# Autodesk Inventor assembly: GE-12022
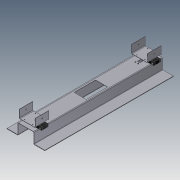
[picture p0: Inventor's stored thumbnail of the model, 180x180]
Saved by Autodesk Inventor 2012 (Build 160160000, 160)
## iProperties
Created: 2011-06-06
Part Number: GE-12022
Document SubType Name: Assembly
Designer: dfoster
Description: Base Assembly, Bridge
Title: Base Assembly, Bridge
Author: dfoster
## Documents named in this file (14)
- C:\Data Folder\FRC 2012 Field\Components\GE-12022.iam
- C:\Data Folder\FRC 2012 Field\Components\GE-12021.ipt
- C:\Data Folder\FRC 2012 Field\Components\PP-00065.ipt
- C:\Data Folder\FRC 2012 Field\Components\GE-12023.ipt
- C:\Data Folder\FRC 2012 Field\Components\GE-12024.ipt
- C:\Data Folder\FRC 2012 Field\Components\GE-12025.ipt
- C:\Data Folder\FRC 2012 Field\Components\HW-00043.0001.ipt
- C:\Data Folder\FRC 2012 Field\Components\HW-00064.ipt
- C:\Data Folder\FRC 2012 Field\Components\HW-00065.ipt
- C:\Data Folder\FRC 2012 Field\Components\HW-00033.ipt
- C:\Data Folder\FRC 2012 Field\Components\GE-12061.ipt
- C:\Data Folder\FRC 2012 Field\Components\HW-00070.ipt
- C:\Data Folder\FRC 2012 Field\Components\HW-00071.ipt
- C:\Data Folder\FRC 2012 Field\Components\GE-12022-01.ipt
## Components (63 placed, 13 different names)
1. GE-12021:1 — Mate:1, Mate:2, Mate:3, Angle:1, Angle:2, Insert:5, Insert:6, Mate:34, Mate:35, Mate:36, Mate:37, Mate:38, Mate:39, Mate:40, Mate:41, Insert:12, Mate:42, Mate:43, Flush:1, Flush:2, Flush:3, Flush:4
2. GE-12061:1 — Mate:34, Mate:35, Mate:36, Insert:11
3. GE-12061:2 — Mate:37, Mate:38, Mate:39, Insert:13
4. GE-12022-01:1 — Mate:42, Flush:2, Flush:4
5. GE-12022-01:2 — Mate:43, Flush:1, Flush:3
6. GE-12023:4 — Mate:4, Mate:5, Mate:6, Mate:11, Mate:12, Mate:13, Mate:14, Angle:1
7. GE-12025:1 — Mate:4, Mate:5, Mate:6, Insert:3, Insert:4
8. GE-12023:2 — Mate:1, Mate:2, Mate:3, Mate:7, Mate:8, Mate:9, Mate:10
9. GE-12024:1 — Mate:15, Mate:16, Mate:17, Mate:18, Mate:31, Mate:33
10. PP-00065:4 — Mate:11, Mate:12, Mate:21, Mate:22
11. PP-00065:3 — Mate:13, Mate:14, Mate:23, Mate:24
12. PP-00065:2 — Mate:7, Mate:8, Mate:19, Mate:20
13. GE-12024:2 — Insert:1, Insert:2, Angle:2, Mate:27, Mate:29
14. PP-00065:5 — Mate:16, Mate:17, Mate:25
15. PP-00065:1 — Mate:9, Mate:10, Mate:25
16. PP-00065:6 — Insert:1, Mate:21, Mate:22, Mate:26
17. PP-00065:7 — Insert:2, Mate:19, Mate:20, Mate:28
18. PP-00065:8 — Mate:15, Mate:18, Mate:23, Mate:24
19. HW-00043.0001:1 — Insert:9
20. HW-00043.0001:2 — Insert:10
21. HW-00043.0001:3 — Insert:7
22. HW-00043.0001:4 — Insert:8
23. HW-00064:1 — Insert:6, Insert:8
24. HW-00064:2 — Insert:5, Insert:7
25. HW-00064:3 — Insert:3, Insert:9
26. HW-00064:4 — Insert:4, Insert:10
27. HW-00065:1 — Mate:26, Mate:27, Mate:30
28. HW-00065:2 — Mate:28, Mate:29, Mate:32
29. HW-00033:1 — Mate:32, Mate:33
30. HW-00033:2 — Mate:30, Mate:31
31. GE-12023:5
32. GE-12025:2
33. GE-12023:6
34. GE-12024:3
35. PP-00065:9
36. PP-00065:10
37. PP-00065:11
38. GE-12024:4
39. PP-00065:12
40. PP-00065:13
41. PP-00065:14
42. PP-00065:15
43. PP-00065:16
44. HW-00043.0001:5
45. HW-00043.0001:6
46. HW-00043.0001:7
47. HW-00043.0001:8
48. HW-00064:5
49. HW-00064:6
50. HW-00064:7
51. HW-00064:8
52. HW-00065:3
53. HW-00065:4
54. HW-00033:3
55. HW-00033:4
56. HW-00070:1 — Mate:40, Mate:41
57. HW-00070:2 — Insert:12
58. HW-00071:1 — Insert:11
59. HW-00071:2 — Insert:13
60. HW-00070:3
61. HW-00070:4
62. HW-00071:3
63. HW-00071:4
## Component patterns: (2 elements, first: GE-12023:4 + GE-12025:1 + GE-12023:2 + GE-12024:1 + PP-00065:4 + PP-00065:3 + PP-00065:2 + GE-12024:2 + PP-00065:5 + PP-00065:1 + PP-00065:6 + PP-00065:7 + PP-00065:8 + HW-00043.0001:1 + HW-00043.0001:2 + HW-00043.0001:3 + HW-00043.0001:4 + HW-00064:1 + HW-00064:2 + HW-00064:3 + HW-00064:4 + HW-00065:1 + HW-00065:2 + HW-00033:1 + HW-00033:2), (2 elements, first: HW-00070:1 + HW-00070:2 + HW-00071:1 + HW-00071:2)
## Relationships (62: Mate 43, Insert 13, Flush 4, Angle 2)
- Mate:1: GE-12021:1 ↔ GE-12023:2
- Mate:2: GE-12021:1 ↔ GE-12023:2
- Mate:3: GE-12021:1 ↔ GE-12023:2
- Mate:4: GE-12023:4 ↔ GE-12025:1
- Mate:5: GE-12023:4 ↔ GE-12025:1
- Mate:6: GE-12023:4 ↔ GE-12025:1
- Mate:7: GE-12023:2 ↔ PP-00065:2
- Mate:8: GE-12023:2 ↔ PP-00065:2
- Mate:9: GE-12023:2 ↔ PP-00065:1
- Mate:10: GE-12023:2 ↔ PP-00065:1
- Mate:11: GE-12023:4 ↔ PP-00065:4
- Mate:12: GE-12023:4 ↔ PP-00065:4
- Mate:13: GE-12023:4 ↔ PP-00065:3
- Mate:14: GE-12023:4 ↔ PP-00065:3
- Mate:15: GE-12024:1 ↔ PP-00065:8
- Mate:16: GE-12024:1 ↔ PP-00065:5
- Mate:17: GE-12024:1 ↔ PP-00065:5
- Mate:18: GE-12024:1 ↔ PP-00065:8
- Insert:1: GE-12024:2 ↔ PP-00065:6
- Insert:2: GE-12024:2 ↔ PP-00065:7
- Mate:19: PP-00065:2 ↔ PP-00065:7
- Mate:20: PP-00065:2 ↔ PP-00065:7
- Mate:21: PP-00065:4 ↔ PP-00065:6
- Mate:22: PP-00065:4 ↔ PP-00065:6
- Mate:23: PP-00065:3 ↔ PP-00065:8
- Mate:24: PP-00065:3 ↔ PP-00065:8
- Mate:25: PP-00065:5 ↔ PP-00065:1
- Angle:1 (0 deg): GE-12021:1 ↔ GE-12023:4
- Angle:2 (0 deg): GE-12021:1 ↔ GE-12024:2
- Insert:3: GE-12025:1 ↔ HW-00064:3
- Insert:4: GE-12025:1 ↔ HW-00064:4
- Insert:5: GE-12021:1 ↔ HW-00064:2
- Insert:6: GE-12021:1 ↔ HW-00064:1
- Insert:7: HW-00043.0001:3 ↔ HW-00064:2
- Insert:8: HW-00043.0001:4 ↔ HW-00064:1
- Insert:9: HW-00043.0001:1 ↔ HW-00064:3
- Insert:10: HW-00043.0001:2 ↔ HW-00064:4
- Mate:26: PP-00065:6 ↔ HW-00065:1
- Mate:27: GE-12024:2 ↔ HW-00065:1
- Mate:28: PP-00065:7 ↔ HW-00065:2
- Mate:29: GE-12024:2 ↔ HW-00065:2
- Mate:30: HW-00065:1 ↔ HW-00033:2
- Mate:31: GE-12024:1 ↔ HW-00033:2
- Mate:32: HW-00065:2 ↔ HW-00033:1
- Mate:33: GE-12024:1 ↔ HW-00033:1
- Mate:34: GE-12021:1 ↔ GE-12061:1
- Mate:35: GE-12021:1 ↔ GE-12061:1
- Mate:36: GE-12021:1 ↔ GE-12061:1
- Mate:37: GE-12021:1 ↔ GE-12061:2
- Mate:38: GE-12021:1 ↔ GE-12061:2
- Mate:39: GE-12021:1 ↔ GE-12061:2
- Mate:40: GE-12021:1 ↔ HW-00070:1
- Mate:41: GE-12021:1 ↔ HW-00070:1
- Insert:11: GE-12061:1 ↔ HW-00071:1
- Insert:12: GE-12021:1 ↔ HW-00070:2
- Insert:13: GE-12061:2 ↔ HW-00071:2
- Mate:42: GE-12021:1 ↔ GE-12022-01:1
- Mate:43: GE-12021:1 ↔ GE-12022-01:2
- Flush:1: GE-12021:1 ↔ GE-12022-01:2
- Flush:2: GE-12021:1 ↔ GE-12022-01:1
- Flush:3: GE-12021:1 ↔ GE-12022-01:2
- Flush:4: GE-12021:1 ↔ GE-12022-01:1
